# Autodesk Inventor assembly: EM Plate
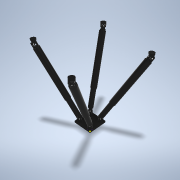
[picture p0: Inventor's stored thumbnail of the model, 180x180]
Saved by Autodesk Inventor 2022 (Build 260153000, 153)
## iProperties
Created: 2022-02-15
Part Number: EM Plate
Document SubType Name: Assembly
Designer: RNG3nius
Author: RNG3nius
## Documents named in this file (8)
- D:\Mason\2021-2022\Capstone\Object Retrieval\EM Plate.iam
- D:\Mason\2021-2022\Capstone\Object Retrieval\EM plate.ipt
- D:\Mason\2021-2022\Capstone\Object Retrieval\joint.ipt
- D:\Mason\2021-2022\Capstone\Object Retrieval\Nut.ipt
- D:\Mason\2021-2022\Capstone\Object Retrieval\shaft.ipt
- D:\Mason\2021-2022\Capstone\Object Retrieval\inner tube.ipt
- D:\Mason\2021-2022\Capstone\Object Retrieval\outer tube.ipt
- D:\Mason\2021-2022\Capstone\Object Retrieval\magnet.ipt
## Components (66 placed, 7 different names)
1. EM plate:1 — Mate:1, Mate:2, Mate:13, Mate:14, Angle:1
2. magnet:1 — Mate:13, Mate:14
3. joint:1 — Mate:1, Mate:2
4. joint:2 — Rotational:1
5. joint:3
6. joint:4
7. Nut:1 — Mate:3, Mate:4
8. joint:5 — Rigid:1, Mate:5, Mate:6
9. Nut:2
10. joint:6
11. Nut:3
12. joint:7
13. Nut:4
14. joint:8
15. inner tube:1 — Mate:5, Mate:6, Mate:7, Mate:8
16. outer tube:1 — Mate:7, Mate:8, Mate:9, Mate:10
17. joint:9 — Mate:9, Mate:10, Rotational:2
18. Nut:5 — Mate:11, Mate:12
19. joint:10 — Rotational:3, Angle:1
20. inner tube:2
21. outer tube:2
22. joint:11
23. Nut:6
24. joint:12
25. inner tube:3
26. outer tube:3
27. joint:13
28. Nut:7
29. joint:14
30. inner tube:4
31. outer tube:4
32. joint:15
33. Nut:8
34. joint:16
35. shaft:1 — Mate:3, Mate:4, Rotational:1
36. shaft:2 — Rigid:1
37. shaft:3
38. shaft:4
39. shaft:5
40. shaft:6
41. shaft:7
42. shaft:8
43. shaft:9
44. shaft:10
45. shaft:11
46. shaft:12
47. shaft:13
48. shaft:14
49. shaft:15
50. shaft:16
51. shaft:17 — Mate:11, Mate:12, Rotational:3
52. shaft:18
53. shaft:19
54. shaft:20 — Rotational:2
55. shaft:21
56. shaft:22
57. shaft:23
58. shaft:24
59. shaft:25
60. shaft:26
61. shaft:27
62. shaft:28
63. shaft:29
64. shaft:30
65. shaft:31
66. shaft:32
## Component patterns: (4 elements, first: joint:1), (4 elements, first: Nut:1 + joint:5), (4 elements, first: inner tube:1 + outer tube:1 + joint:9 + Nut:5 + joint:10), (4 elements, first: shaft:1), Component Pattern 2:2 (4 elements), Component Pattern 2:3 (4 elements), Component Pattern 2:4 (4 elements), (4 elements, first: shaft:17), Component Pattern 4:2 (4 elements), Component Pattern 4:3 (4 elements), Component Pattern 4:4 (4 elements)
## Relationships (19: Mate 14, RevoluteJoint 3, WeldJoint 1, Angle 1)
- Mate:1: EM plate:1 ↔ joint:1
- Mate:2: EM plate:1 ↔ joint:1
- Mate:3: Nut:1 ↔ shaft:1
- Mate:4: Nut:1 ↔ shaft:1
- Rigid:1 [WeldJoint]: joint:5 ↔ shaft:2
- Rotational:1 [RevoluteJoint]: joint:2 ↔ shaft:1
- Mate:5: joint:5 ↔ inner tube:1
- Mate:6: joint:5 ↔ inner tube:1
- Mate:7: inner tube:1 ↔ outer tube:1
- Mate:8: inner tube:1 ↔ outer tube:1
- Mate:9: outer tube:1 ↔ joint:9
- Mate:10: outer tube:1 ↔ joint:9
- Mate:11: Nut:5 ↔ shaft:17
- Mate:12: Nut:5 ↔ shaft:17
- Rotational:2 [RevoluteJoint]: joint:9 ↔ shaft:20
- Rotational:3 [RevoluteJoint]: joint:10 ↔ shaft:17
- Mate:13: EM plate:1 ↔ magnet:1
- Mate:14: EM plate:1 ↔ magnet:1
- Angle:1 (0 deg): EM plate:1 ↔ joint:10
